# Autodesk Inventor assembly: robot_hand
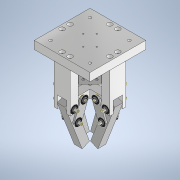
[picture p0: Inventor's stored thumbnail of the model, 180x180]
Saved by Autodesk Inventor 2021 (Build 250183000, 183)
## iProperties
Created: 2021-10-20
Part Number: robot_hand
Document SubType Name: Assembly
Designer: ryusei
Author: ryusei
## Documents named in this file (16)
- C:\Users\ryusei\Documents\Inventor\robot_design3\完成版\robot_hand.iam
- C:\Users\ryusei\Documents\Inventor\robot_design3\完成版\部品\ハンド土台.ipt
- C:\Users\ryusei\Documents\Inventor\robot_design3\完成版\部品\ハンド支え.ipt
- C:\Users\ryusei\Documents\Inventor\robot_design3\完成版\部品\シリンダ固定.ipt
- C:\Users\ryusei\Documents\Inventor\robot_design3\完成版\部品\MBDA6×15_シリンダコガネイ\伸びるやつ１.ipt
- C:\Users\ryusei\Documents\Inventor\robot_design3\完成版\部品\MBDA6×15_シリンダコガネイ\伸びるやつ2.ipt
- C:\Users\ryusei\Documents\Inventor\robot_design3\完成版\部品\MBDA6×15_シリンダコガネイ\本体.ipt
- C:\Users\ryusei\Documents\Inventor\robot_design3\完成版\部品\シリンダ先端パーツ.ipt
- C:\Users\ryusei\Documents\Inventor\robot_design3\完成版\部品\ステンレス平行ピンΦ3h7_30.ipt
- C:\Users\ryusei\Documents\Inventor\robot_design3\完成版\部品\ハンド10×10×60.ipt
- C:\Users\ryusei\Documents\Inventor\robot_design3\完成版\部品\MF63ZZ_ベアリング.ipt
- C:\Users\ryusei\Documents\Inventor\robot_design3\完成版\部品\ステンレス平行ピンΦ3h7_25.ipt
- C:\Users\ryusei\Documents\Inventor\robot_design3\完成版\部品\ステンレス平行ピンΦ3h7_18.ipt
- C:\Users\ryusei\Documents\Inventor\robot_design3\完成版\部品\樹脂ワッシャ(ポリスライダー).ipt
- C:\Users\ryusei\Documents\Inventor\robot_design3\完成版\部品\リンク26×6×2.ipt
- C:\Users\ryusei\Documents\Inventor\robot_design3\完成版\部品\Φ3軸用プッシュナット.ipt
## Components (107 placed, 15 different names)
1. ハンド土台:1 — 挿入:116, 挿入:117, 挿入:118, 挿入:119, 挿入:120, 挿入:121, 挿入:122, 挿入:123, 挿入:131, 挿入:132, 挿入:133, 挿入:134, 挿入:135
2. ハンド支え:1 — 挿入:22, 挿入:107, 挿入:108, 挿入:116, 挿入:117, 挿入:131, 角度:1
3. ハンド支え:2 — 挿入:21, 挿入:103, 挿入:105, 挿入:122, 挿入:123
4. ハンド支え:3 — 挿入:23, 挿入:110, 挿入:112, 挿入:118, 挿入:119
5. ハンド支え:4 — 挿入:20, 挿入:101, 挿入:115, 挿入:120, 挿入:121
6. シリンダ固定:1 — 挿入:14, 挿入:15, 挿入:134, 挿入:135
7. 伸びるやつ１:1 — 挿入:13, メイト:1, 円柱状:1
8. 伸びるやつ2:1 — 挿入:13, 挿入:19
9. 本体:1 — 挿入:14, 挿入:15, 挿入:17, メイト:1, 円柱状:1
10. シリンダ固定:2 — 挿入:17, 挿入:132, 挿入:133
11. シリンダ先端パーツ:1 — 挿入:19, 挿入:28, 挿入:29, 挿入:30, 挿入:31, 挿入:32, 挿入:33, 挿入:34, 挿入:35, 挿入:128, 挿入:129, 挿入:130, 角度:1
12. ステンレス平行ピンΦ3h7_30:1 — 挿入:22, 挿入:49
13. ステンレス平行ピンΦ3h7_30:2 — 挿入:21, 挿入:50
14. ステンレス平行ピンΦ3h7_30:3 — 挿入:23, 挿入:48
15. ステンレス平行ピンΦ3h7_30:4 — 挿入:20, 挿入:51
16. ハンド10×10×60:1 — 挿入:40, 挿入:41, 挿入:46, 挿入:47
17. ハンド10×10×60:2 — 挿入:38, 挿入:39, 挿入:44, 挿入:45
18. ハンド10×10×60:3 — 挿入:36, 挿入:37, 挿入:42, 挿入:43
19. ハンド10×10×60:4 — 挿入:24, 挿入:25, 挿入:26, 挿入:27
20. MF63ZZ_ベアリング:1 — 挿入:31, 挿入:59, 挿入:62, 挿入:128
21. MF63ZZ_ベアリング:2 — 挿入:30, 挿入:63, 挿入:130
22. MF63ZZ_ベアリング:3 — 挿入:28, 挿入:56, 挿入:60
23. MF63ZZ_ベアリング:4 — 挿入:29, 挿入:57, 挿入:61
24. MF63ZZ_ベアリング:5 — 挿入:33, 挿入:58, 挿入:66
25. MF63ZZ_ベアリング:6 — 挿入:35, 挿入:65
26. MF63ZZ_ベアリング:7 — 挿入:32, 挿入:67
27. MF63ZZ_ベアリング:8 — 挿入:34, 挿入:64, 挿入:129
28. MF63ZZ_ベアリング:9 — 挿入:36, 挿入:76
29. MF63ZZ_ベアリング:10 — 挿入:38, 挿入:75
30. MF63ZZ_ベアリング:11 — 挿入:39, 挿入:51, 挿入:74
31. MF63ZZ_ベアリング:12 — 挿入:37, 挿入:50, 挿入:77
32. MF63ZZ_ベアリング:13 — 挿入:45, 挿入:53, 挿入:72
33. MF63ZZ_ベアリング:14 — 挿入:47, 挿入:55, 挿入:80
34. MF63ZZ_ベアリング:15 — 挿入:40, 挿入:82
35. MF63ZZ_ベアリング:16 — 挿入:41, 挿入:83
36. MF63ZZ_ベアリング:17 — 挿入:42, 挿入:79
37. MF63ZZ_ベアリング:18 — 挿入:27, 挿入:48, 挿入:69
38. MF63ZZ_ベアリング:19 — 挿入:46, 挿入:49, 挿入:81
39. MF63ZZ_ベアリング:20 — 挿入:43, 挿入:54, 挿入:78
40. MF63ZZ_ベアリング:21 — 挿入:44, 挿入:73
41. MF63ZZ_ベアリング:22 — 挿入:25, 挿入:71
42. MF63ZZ_ベアリング:23 — 挿入:24, 挿入:70
43. MF63ZZ_ベアリング:24 — 挿入:26, 挿入:52, 挿入:68
44. ステンレス平行ピンΦ3h7_25:1 — 挿入:55
45. ステンレス平行ピンΦ3h7_25:2 — 挿入:54
46. ステンレス平行ピンΦ3h7_25:3 — 挿入:53
47. ステンレス平行ピンΦ3h7_25:4 — 挿入:52
48. ステンレス平行ピンΦ3h7_18:1 — 挿入:56
49. ステンレス平行ピンΦ3h7_18:2 — 挿入:57
50. ステンレス平行ピンΦ3h7_18:3 — 挿入:59
51. ステンレス平行ピンΦ3h7_18:4 — 挿入:58
52. 樹脂ワッシャ(ポリスライダー):1 — 挿入:68, 挿入:86
53. 樹脂ワッシャ(ポリスライダー):2 — 挿入:71, 挿入:91
54. 樹脂ワッシャ(ポリスライダー):3 — 挿入:69
55. 樹脂ワッシャ(ポリスライダー):4 — 挿入:70
56. 樹脂ワッシャ(ポリスライダー):5 — 挿入:61, 挿入:138
57. 樹脂ワッシャ(ポリスライダー):6 — 挿入:67, 挿入:139
58. 樹脂ワッシャ(ポリスライダー):7 — 挿入:66, 挿入:140
59. 樹脂ワッシャ(ポリスライダー):8 — 挿入:65, 挿入:141
60. 樹脂ワッシャ(ポリスライダー):9 — 挿入:64, 挿入:142
61. 樹脂ワッシャ(ポリスライダー):10 — 挿入:62, 挿入:143
62. 樹脂ワッシャ(ポリスライダー):11 — 挿入:63, 挿入:137
63. 樹脂ワッシャ(ポリスライダー):12 — 挿入:60, 挿入:136
64. 樹脂ワッシャ(ポリスライダー):13 — 挿入:74
65. 樹脂ワッシャ(ポリスライダー):14 — 挿入:75, 挿入:90
66. 樹脂ワッシャ(ポリスライダー):15 — 挿入:73
67. 樹脂ワッシャ(ポリスライダー):16 — 挿入:72, 挿入:87
68. 樹脂ワッシャ(ポリスライダー):17 — 挿入:78, 挿入:88
69. 樹脂ワッシャ(ポリスライダー):18 — 挿入:79
70. 樹脂ワッシャ(ポリスライダー):19 — 挿入:76, 挿入:84
71. 樹脂ワッシャ(ポリスライダー):20 — 挿入:77
72. 樹脂ワッシャ(ポリスライダー):21 — 挿入:83
73. 樹脂ワッシャ(ポリスライダー):22 — 挿入:82, 挿入:89
74. 樹脂ワッシャ(ポリスライダー):23 — 挿入:80, 挿入:85
75. 樹脂ワッシャ(ポリスライダー):24 — 挿入:81
76. リンク26×6×2:1 — 挿入:85, 挿入:109, 挿入:136, 挿入:150
77. リンク26×6×2:2 — 挿入:84, 挿入:104, 挿入:143, 挿入:148
78. リンク26×6×2:3 — 挿入:89, 挿入:106, 挿入:137, 挿入:149
79. リンク26×6×2:4 — 挿入:90, 挿入:100, 挿入:141, 挿入:146
80. リンク26×6×2:5 — 挿入:86, 挿入:111, 挿入:138, 挿入:151
81. リンク26×6×2:6 — 挿入:87, 挿入:114, 挿入:140, 挿入:145
82. リンク26×6×2:7 — 挿入:91, 挿入:113, 挿入:139, 挿入:144
83. リンク26×6×2:8 — 挿入:88, 挿入:102, 挿入:142, 挿入:147
84. Φ3軸用プッシュナット:1 — 挿入:100
85. Φ3軸用プッシュナット:2 — 挿入:101
86. Φ3軸用プッシュナット:3 — 挿入:114
87. Φ3軸用プッシュナット:4 — 挿入:115
88. Φ3軸用プッシュナット:5 — 挿入:113
89. Φ3軸用プッシュナット:6 — 挿入:112
90. Φ3軸用プッシュナット:7 — 挿入:111
91. Φ3軸用プッシュナット:8 — 挿入:110
92. Φ3軸用プッシュナット:9 — 挿入:108
93. Φ3軸用プッシュナット:10 — 挿入:109
94. Φ3軸用プッシュナット:11 — 挿入:107
95. Φ3軸用プッシュナット:12 — 挿入:106
96. Φ3軸用プッシュナット:13 — 挿入:104
97. Φ3軸用プッシュナット:14 — 挿入:105
98. Φ3軸用プッシュナット:15 — 挿入:102
99. Φ3軸用プッシュナット:16 — 挿入:103
100. Φ3軸用プッシュナット:17 — 挿入:150
101. Φ3軸用プッシュナット:18 — 挿入:151
102. Φ3軸用プッシュナット:19 — 挿入:144
103. Φ3軸用プッシュナット:20 — 挿入:145
104. Φ3軸用プッシュナット:21 — 挿入:146
105. Φ3軸用プッシュナット:22 — 挿入:147
106. Φ3軸用プッシュナット:23 — 挿入:149
107. Φ3軸用プッシュナット:24 — 挿入:148
## Relationships (128: Insert 125, Mate 1, CylindricalJoint 1, Angle 1)
- 挿入:13 [Insert]: 伸びるやつ１:1 ↔ 伸びるやつ2:1
- 挿入:14 [Insert]: シリンダ固定:1 ↔ 本体:1
- 挿入:15 [Insert]: シリンダ固定:1 ↔ 本体:1
- 挿入:17 [Insert]: 本体:1 ↔ シリンダ固定:2
- メイト:1 [Mate]: 伸びるやつ１:1 ↔ 本体:1
- 挿入:19 [Insert]: 伸びるやつ2:1 ↔ シリンダ先端パーツ:1
- 挿入:20 [Insert] (-5 mm): ハンド支え:4 ↔ ステンレス平行ピンΦ3h7_30:4
- 挿入:21 [Insert] (-5 mm): ハンド支え:2 ↔ ステンレス平行ピンΦ3h7_30:2
- 挿入:22 [Insert] (-5 mm): ハンド支え:1 ↔ ステンレス平行ピンΦ3h7_30:1
- 挿入:23 [Insert] (-5 mm): ハンド支え:3 ↔ ステンレス平行ピンΦ3h7_30:3
- 挿入:24 [Insert]: ハンド10×10×60:4 ↔ MF63ZZ_ベアリング:23
- 挿入:25 [Insert]: ハンド10×10×60:4 ↔ MF63ZZ_ベアリング:22
- 挿入:26 [Insert]: ハンド10×10×60:4 ↔ MF63ZZ_ベアリング:24
- 挿入:27 [Insert]: ハンド10×10×60:4 ↔ MF63ZZ_ベアリング:18
- 挿入:28 [Insert]: シリンダ先端パーツ:1 ↔ MF63ZZ_ベアリング:3
- 挿入:29 [Insert]: シリンダ先端パーツ:1 ↔ MF63ZZ_ベアリング:4
- 挿入:30 [Insert]: シリンダ先端パーツ:1 ↔ MF63ZZ_ベアリング:2
- 挿入:31 [Insert]: シリンダ先端パーツ:1 ↔ MF63ZZ_ベアリング:1
- 挿入:32 [Insert]: シリンダ先端パーツ:1 ↔ MF63ZZ_ベアリング:7
- 挿入:33 [Insert]: シリンダ先端パーツ:1 ↔ MF63ZZ_ベアリング:5
- 挿入:34 [Insert]: シリンダ先端パーツ:1 ↔ MF63ZZ_ベアリング:8
- 挿入:35 [Insert]: シリンダ先端パーツ:1 ↔ MF63ZZ_ベアリング:6
- 挿入:36 [Insert]: ハンド10×10×60:3 ↔ MF63ZZ_ベアリング:9
- 挿入:37 [Insert]: ハンド10×10×60:3 ↔ MF63ZZ_ベアリング:12
- 挿入:38 [Insert]: ハンド10×10×60:2 ↔ MF63ZZ_ベアリング:10
- 挿入:39 [Insert]: ハンド10×10×60:2 ↔ MF63ZZ_ベアリング:11
- 挿入:40 [Insert]: ハンド10×10×60:1 ↔ MF63ZZ_ベアリング:15
- 挿入:41 [Insert]: ハンド10×10×60:1 ↔ MF63ZZ_ベアリング:16
- 挿入:42 [Insert]: ハンド10×10×60:3 ↔ MF63ZZ_ベアリング:17
- 挿入:43 [Insert]: ハンド10×10×60:3 ↔ MF63ZZ_ベアリング:20
- 挿入:44 [Insert]: ハンド10×10×60:2 ↔ MF63ZZ_ベアリング:21
- 挿入:45 [Insert]: ハンド10×10×60:2 ↔ MF63ZZ_ベアリング:13
- 挿入:46 [Insert]: ハンド10×10×60:1 ↔ MF63ZZ_ベアリング:19
- 挿入:47 [Insert]: ハンド10×10×60:1 ↔ MF63ZZ_ベアリング:14
- 挿入:48 [Insert] (9.4 mm): ステンレス平行ピンΦ3h7_30:3 ↔ MF63ZZ_ベアリング:18
- 挿入:49 [Insert] (9.4 mm): ステンレス平行ピンΦ3h7_30:1 ↔ MF63ZZ_ベアリング:19
- 挿入:50 [Insert] (9.4 mm): ステンレス平行ピンΦ3h7_30:2 ↔ MF63ZZ_ベアリング:12
- 挿入:51 [Insert] (9.4 mm): ステンレス平行ピンΦ3h7_30:4 ↔ MF63ZZ_ベアリング:11
- 挿入:52 [Insert] (-6.9 mm): MF63ZZ_ベアリング:24 ↔ ステンレス平行ピンΦ3h7_25:4
- 挿入:53 [Insert] (-6.9 mm): MF63ZZ_ベアリング:13 ↔ ステンレス平行ピンΦ3h7_25:3
- 挿入:54 [Insert] (-6.9 mm): MF63ZZ_ベアリング:20 ↔ ステンレス平行ピンΦ3h7_25:2
- 挿入:55 [Insert] (-6.9 mm): MF63ZZ_ベアリング:14 ↔ ステンレス平行ピンΦ3h7_25:1
- 挿入:56 [Insert] (-4.4 mm): MF63ZZ_ベアリング:3 ↔ ステンレス平行ピンΦ3h7_18:1
- 挿入:57 [Insert] (-4.4 mm): MF63ZZ_ベアリング:4 ↔ ステンレス平行ピンΦ3h7_18:2
- 挿入:58 [Insert] (-4.4 mm): MF63ZZ_ベアリング:5 ↔ ステンレス平行ピンΦ3h7_18:4
- 挿入:59 [Insert] (-4.4 mm): MF63ZZ_ベアリング:1 ↔ ステンレス平行ピンΦ3h7_18:3
- 挿入:60 [Insert]: MF63ZZ_ベアリング:3 ↔ 樹脂ワッシャ(ポリスライダー):12
- 挿入:61 [Insert]: MF63ZZ_ベアリング:4 ↔ 樹脂ワッシャ(ポリスライダー):5
- 挿入:62 [Insert]: MF63ZZ_ベアリング:1 ↔ 樹脂ワッシャ(ポリスライダー):10
- 挿入:63 [Insert]: MF63ZZ_ベアリング:2 ↔ 樹脂ワッシャ(ポリスライダー):11
- 挿入:64 [Insert]: MF63ZZ_ベアリング:8 ↔ 樹脂ワッシャ(ポリスライダー):9
- 挿入:65 [Insert]: MF63ZZ_ベアリング:6 ↔ 樹脂ワッシャ(ポリスライダー):8
- 挿入:66 [Insert]: MF63ZZ_ベアリング:5 ↔ 樹脂ワッシャ(ポリスライダー):7
- 挿入:67 [Insert]: MF63ZZ_ベアリング:7 ↔ 樹脂ワッシャ(ポリスライダー):6
- 挿入:68 [Insert]: MF63ZZ_ベアリング:24 ↔ 樹脂ワッシャ(ポリスライダー):1
- 挿入:69 [Insert]: MF63ZZ_ベアリング:18 ↔ 樹脂ワッシャ(ポリスライダー):3
- 挿入:70 [Insert]: MF63ZZ_ベアリング:23 ↔ 樹脂ワッシャ(ポリスライダー):4
- 挿入:71 [Insert]: MF63ZZ_ベアリング:22 ↔ 樹脂ワッシャ(ポリスライダー):2
- 挿入:72 [Insert]: MF63ZZ_ベアリング:13 ↔ 樹脂ワッシャ(ポリスライダー):16
- 挿入:73 [Insert]: MF63ZZ_ベアリング:21 ↔ 樹脂ワッシャ(ポリスライダー):15
- 挿入:74 [Insert]: MF63ZZ_ベアリング:11 ↔ 樹脂ワッシャ(ポリスライダー):13
- 挿入:75 [Insert]: MF63ZZ_ベアリング:10 ↔ 樹脂ワッシャ(ポリスライダー):14
- 挿入:76 [Insert]: MF63ZZ_ベアリング:9 ↔ 樹脂ワッシャ(ポリスライダー):19
- 挿入:77 [Insert]: MF63ZZ_ベアリング:12 ↔ 樹脂ワッシャ(ポリスライダー):20
- 挿入:78 [Insert]: MF63ZZ_ベアリング:20 ↔ 樹脂ワッシャ(ポリスライダー):17
- 挿入:79 [Insert]: MF63ZZ_ベアリング:17 ↔ 樹脂ワッシャ(ポリスライダー):18
- 挿入:80 [Insert]: MF63ZZ_ベアリング:14 ↔ 樹脂ワッシャ(ポリスライダー):23
- 挿入:81 [Insert]: MF63ZZ_ベアリング:19 ↔ 樹脂ワッシャ(ポリスライダー):24
- 挿入:82 [Insert]: MF63ZZ_ベアリング:15 ↔ 樹脂ワッシャ(ポリスライダー):22
- 挿入:83 [Insert]: MF63ZZ_ベアリング:16 ↔ 樹脂ワッシャ(ポリスライダー):21
- 挿入:84 [Insert]: 樹脂ワッシャ(ポリスライダー):19 ↔ リンク26×6×2:2
- 挿入:85 [Insert]: 樹脂ワッシャ(ポリスライダー):23 ↔ リンク26×6×2:1
- 挿入:86 [Insert]: 樹脂ワッシャ(ポリスライダー):1 ↔ リンク26×6×2:5
- 挿入:87 [Insert]: 樹脂ワッシャ(ポリスライダー):16 ↔ リンク26×6×2:6
- 挿入:88 [Insert]: 樹脂ワッシャ(ポリスライダー):17 ↔ リンク26×6×2:8
- 挿入:89 [Insert]: 樹脂ワッシャ(ポリスライダー):22 ↔ リンク26×6×2:3
- 挿入:90 [Insert]: 樹脂ワッシャ(ポリスライダー):14 ↔ リンク26×6×2:4
- 挿入:91 [Insert]: 樹脂ワッシャ(ポリスライダー):2 ↔ リンク26×6×2:7
- 円柱状:1 [CylindricalJoint]: 伸びるやつ１:1 ↔ 本体:1
- 挿入:100 [Insert]: リンク26×6×2:4 ↔ Φ3軸用プッシュナット:1
- 挿入:101 [Insert]: ハンド支え:4 ↔ Φ3軸用プッシュナット:2
- 挿入:102 [Insert]: リンク26×6×2:8 ↔ Φ3軸用プッシュナット:15
- 挿入:103 [Insert]: ハンド支え:2 ↔ Φ3軸用プッシュナット:16
- 挿入:104 [Insert]: リンク26×6×2:2 ↔ Φ3軸用プッシュナット:13
- 挿入:105 [Insert]: ハンド支え:2 ↔ Φ3軸用プッシュナット:14
- 挿入:106 [Insert]: リンク26×6×2:3 ↔ Φ3軸用プッシュナット:12
- 挿入:107 [Insert]: ハンド支え:1 ↔ Φ3軸用プッシュナット:11
- 挿入:108 [Insert]: ハンド支え:1 ↔ Φ3軸用プッシュナット:9
- 挿入:109 [Insert]: リンク26×6×2:1 ↔ Φ3軸用プッシュナット:10
- 挿入:110 [Insert]: ハンド支え:3 ↔ Φ3軸用プッシュナット:8
- 挿入:111 [Insert]: リンク26×6×2:5 ↔ Φ3軸用プッシュナット:7
- 挿入:112 [Insert]: ハンド支え:3 ↔ Φ3軸用プッシュナット:6
- 挿入:113 [Insert]: リンク26×6×2:7 ↔ Φ3軸用プッシュナット:5
- 挿入:114 [Insert]: リンク26×6×2:6 ↔ Φ3軸用プッシュナット:3
- 挿入:115 [Insert]: ハンド支え:4 ↔ Φ3軸用プッシュナット:4
- 挿入:116 [Insert]: ハンド土台:1 ↔ ハンド支え:1
- 挿入:117 [Insert]: ハンド土台:1 ↔ ハンド支え:1
- 挿入:118 [Insert]: ハンド土台:1 ↔ ハンド支え:3
- 挿入:119 [Insert]: ハンド土台:1 ↔ ハンド支え:3
- 挿入:120 [Insert]: ハンド土台:1 ↔ ハンド支え:4
- 挿入:121 [Insert]: ハンド土台:1 ↔ ハンド支え:4
- 挿入:122 [Insert]: ハンド土台:1 ↔ ハンド支え:2
- 挿入:123 [Insert]: ハンド土台:1 ↔ ハンド支え:2
- 挿入:128 [Insert]: シリンダ先端パーツ:1 ↔ MF63ZZ_ベアリング:1
- 挿入:129 [Insert]: シリンダ先端パーツ:1 ↔ MF63ZZ_ベアリング:8
- 挿入:130 [Insert]: シリンダ先端パーツ:1 ↔ MF63ZZ_ベアリング:2
- 挿入:131 [Insert]: ハンド土台:1 ↔ ハンド支え:1
- 挿入:132 [Insert]: ハンド土台:1 ↔ シリンダ固定:2
- 挿入:133 [Insert]: ハンド土台:1 ↔ シリンダ固定:2
- 挿入:134 [Insert]: ハンド土台:1 ↔ シリンダ固定:1
- 挿入:135 [Insert]: ハンド土台:1 ↔ シリンダ固定:1
- 角度:1 [Angle] (0 deg): ハンド支え:1 ↔ シリンダ先端パーツ:1
- 挿入:136 [Insert]: 樹脂ワッシャ(ポリスライダー):12 ↔ リンク26×6×2:1
- 挿入:137 [Insert]: 樹脂ワッシャ(ポリスライダー):11 ↔ リンク26×6×2:3
- 挿入:138 [Insert]: 樹脂ワッシャ(ポリスライダー):5 ↔ リンク26×6×2:5
- 挿入:139 [Insert]: 樹脂ワッシャ(ポリスライダー):6 ↔ リンク26×6×2:7
- 挿入:140 [Insert]: 樹脂ワッシャ(ポリスライダー):7 ↔ リンク26×6×2:6
- 挿入:141 [Insert]: 樹脂ワッシャ(ポリスライダー):8 ↔ リンク26×6×2:4
- 挿入:142 [Insert]: 樹脂ワッシャ(ポリスライダー):9 ↔ リンク26×6×2:8
- 挿入:143 [Insert]: 樹脂ワッシャ(ポリスライダー):10 ↔ リンク26×6×2:2
- 挿入:144 [Insert]: リンク26×6×2:7 ↔ Φ3軸用プッシュナット:19
- 挿入:145 [Insert]: リンク26×6×2:6 ↔ Φ3軸用プッシュナット:20
- 挿入:146 [Insert]: リンク26×6×2:4 ↔ Φ3軸用プッシュナット:21
- 挿入:147 [Insert]: リンク26×6×2:8 ↔ Φ3軸用プッシュナット:22
- 挿入:148 [Insert]: リンク26×6×2:2 ↔ Φ3軸用プッシュナット:24
- 挿入:149 [Insert]: リンク26×6×2:3 ↔ Φ3軸用プッシュナット:23
- 挿入:150 [Insert]: リンク26×6×2:1 ↔ Φ3軸用プッシュナット:17
- 挿入:151 [Insert]: リンク26×6×2:5 ↔ Φ3軸用プッシュナット:18
